# Autodesk Inventor assembly: Gear Assembly
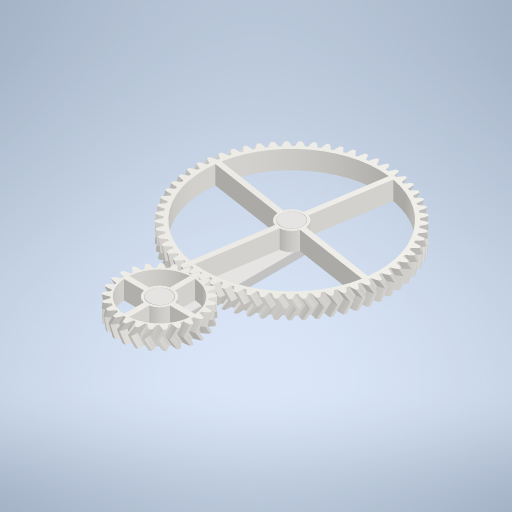
[picture p0: Inventor's stored thumbnail of the model, 512x512]
Saved by Autodesk Inventor 2024.3 (Build 283343000, 343)
## iProperties
Created: 2024-11-06
Part Number: Gear Assembly
Document SubType Name: Assembly
Designer: wszaf
Author: wszaf
## Documents named in this file (9)
- C:\Users\wszaf\Desktop\Pulpit\3D Printing\Test Prints\Gear Module\Gear Assembly.iam
- C:\Users\wszaf\Desktop\Pulpit\3D Printing\Test Prints\Gear Module\Base Diameter 8 Lenght 50.ipt
- C:\Users\wszaf\Desktop\Pulpit\3D Printing\Test Prints\Gear Module\Gear Assembly\Design Accelerator\Spur Gears1.iam
- C:\Users\wszaf\Desktop\Pulpit\3D Printing\Test Prints\Gear Module\Gear Assembly\Design Accelerator\Spur Gears2.iam
- C:\Users\wszaf\Desktop\Pulpit\3D Printing\Test Prints\Gear Module\Gear Assembly\Design Accelerator\Spur Gears3.iam
- C:\Users\wszaf\Desktop\Pulpit\3D Printing\Test Prints\Gear Module\Gear Assembly\Design Accelerator\Spur Gears4.iam
- C:\Users\wszaf\Desktop\Pulpit\3D Printing\Test Prints\Gear Module\Gear Assembly\Design Accelerator\Spur Gears5.iam
- C:\Users\wszaf\Desktop\Pulpit\3D Printing\Test Prints\Gear Module\Gear Assembly\Design Accelerator\Spur Gears6.iam
- C:\Users\wszaf\Desktop\Pulpit\3D Printing\Test Prints\Gear Module\Gear Assembly\Design Accelerator\Spur Gears7.iam
## Components (8 placed, 8 different names)
1. Base Diameter 8 Lenght 50:1 — Mate:1, Flush:1, Mate:2, Flush:2, Mate:3, Flush:3, Mate:4, Flush:4, Mate:5, Flush:5, Mate:6, Flush:6, Mate:7, Flush:7, Mate:8, Flush:8, Mate:9, Flush:9, Mate:10, Flush:10, Mate:17, Mate:18, Mate:19, Mate:20, Mate:21, Flush:11, Mate:22, Flush:12
2. Module 1 [sub-assembly] — Mate:1, Flush:1, Mate:2, Flush:2
3. Module 2 [sub-assembly] — Mate:3, Flush:3, Mate:4, Flush:4
4. Module 0.5 [sub-assembly] — Mate:5, Flush:5, Mate:6, Flush:6
5. Module 3 [sub-assembly] — Mate:7, Flush:7, Mate:8, Flush:8
6. Module 0.7 [sub-assembly] — Mate:9, Flush:9, Mate:10, Flush:10
7. Module 1 Single Helix [sub-assembly] — Mate:17, Mate:18, Mate:19, Mate:20
8. Module1 Double Helix Half [sub-assembly] — Mate:21, Flush:11, Mate:22, Flush:12
## Relationships (28: Mate 16, Flush 12)
- Mate:1: Base Diameter 8 Lenght 50:1 ↔ Module 1
- Flush:1: Base Diameter 8 Lenght 50:1 ↔ Module 1
- Mate:2: Base Diameter 8 Lenght 50:1 ↔ Module 1
- Flush:2: Base Diameter 8 Lenght 50:1 ↔ Module 1
- Mate:3: Base Diameter 8 Lenght 50:1 ↔ Module 2
- Flush:3: Base Diameter 8 Lenght 50:1 ↔ Module 2
- Mate:4: Base Diameter 8 Lenght 50:1 ↔ Module 2
- Flush:4: Base Diameter 8 Lenght 50:1 ↔ Module 2
- Mate:5: Base Diameter 8 Lenght 50:1 ↔ Module 0.5
- Flush:5: Base Diameter 8 Lenght 50:1 ↔ Module 0.5
- Mate:6: Base Diameter 8 Lenght 50:1 ↔ Module 0.5
- Flush:6: Base Diameter 8 Lenght 50:1 ↔ Module 0.5
- Mate:7: Base Diameter 8 Lenght 50:1 ↔ Module 3
- Flush:7: Base Diameter 8 Lenght 50:1 ↔ Module 3
- Mate:8: Base Diameter 8 Lenght 50:1 ↔ Module 3
- Flush:8: Base Diameter 8 Lenght 50:1 ↔ Module 3
- Mate:9: Base Diameter 8 Lenght 50:1 ↔ Module 0.7
- Flush:9: Base Diameter 8 Lenght 50:1 ↔ Module 0.7
- Mate:10: Base Diameter 8 Lenght 50:1 ↔ Module 0.7
- Flush:10: Base Diameter 8 Lenght 50:1 ↔ Module 0.7
- Mate:17: Base Diameter 8 Lenght 50:1 ↔ Module 1 Single Helix
- Mate:18: Base Diameter 8 Lenght 50:1 ↔ Module 1 Single Helix
- Mate:19: Base Diameter 8 Lenght 50:1 ↔ Module 1 Single Helix
- Mate:20: Base Diameter 8 Lenght 50:1 ↔ Module 1 Single Helix
- Mate:21: Base Diameter 8 Lenght 50:1 ↔ Module1 Double Helix Half
- Flush:11: Base Diameter 8 Lenght 50:1 ↔ Module1 Double Helix Half
- Mate:22: Base Diameter 8 Lenght 50:1 ↔ Module1 Double Helix Half
- Flush:12: Base Diameter 8 Lenght 50:1 ↔ Module1 Double Helix Half
